# Autodesk Inventor assembly: 0.3rd Lawette - V3.0
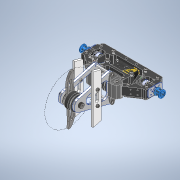
[picture p0: Inventor's stored thumbnail of the model, 180x180]
Saved by Autodesk Inventor 2022.1 (Build 261234020, 234B)
## iProperties
Created: 2022-05-21
Part Number: 0.3rd Lawette - V3.0
Document SubType Name: Assembly
Designer: Nathan Cai
Mass: 1280.13 g
Surface Area: 3794.37 cm^2
Volume: 778.123 cm^3
Density: 1.64515 g/cm^3
Author: Nathan Cai
## Documents named in this file (24)
- D:\Inventor\0.3rd Lawette - V3.0\0.3rd Lawette - V3.0.iam
- D:\Inventor\0.3rd Lawette - V3.0\RR Brushless\RR-Brushless-Planetary.iam
- D:\Inventor\0.3rd Lawette - V3.0\Tattu 4S 650mah\Tattu 650mah 4S.iam
- D:\Inventor\0.3rd Lawette - V3.0\BL20A.ipt
- D:\Inventor\0.3rd Lawette - V3.0\Talon 25A ESC.ipt
- D:\Inventor\0.3rd Lawette - V3.0\Receiver (FrSky RX6R).ipt
- D:\Inventor\0.3rd Lawette - V3.0\Fingertech Power Switch\Fingertech Mini Power Switch.iam
- D:\Inventor\0.3rd Lawette - V3.0\Weapon Assembly.iam
- D:\Inventor\0.3rd Lawette - V3.0\Hubs (Fingertech Twisthub).ipt
- D:\Inventor\0.3rd Lawette - V3.0\Chassis.ipt
- D:\Inventor\0.3rd Lawette - V3.0\Tires (Fingertech Foam Wheels).ipt
- D:\Inventor\0.3rd Lawette - V3.0\Standoff 1.5in.ipt
- D:\Inventor\0.3rd Lawette - V3.0\Cover (Inner).ipt
- D:\Inventor\0.3rd Lawette - V3.0\Cover (Inner Top).ipt
- C:\Users\NCai2\Documents\Inventor\Content Center Files\R2022\en-US\ANSI B18.6.3(27)\ANSI B18.6.3 - 6-32 UNC - 0.5(11).ipt
- D:\Inventor\0.3rd Lawette - V3.0\Cover (Outer).ipt
- C:\Users\NCai2\Documents\Inventor\Content Center Files\R2022\en-US\ANSI B18.6.3(27)\ANSI B18.6.3 - 6-32 UNC - 0.375(11).ipt
- C:\Users\NCai2\Documents\Inventor\Content Center Files\R2022\en-US\ANSI B18.6.3(27)\ANSI B18.6.3 - 6-32 UNC - 0.4375(11).ipt
- C:\Users\NCai2\Documents\Inventor\Content Center Files\R2022\en-US\SAE J773b\SAE J773b - No. 6. SAE Type L. Regular.ipt
- D:\Inventor\0.3rd Lawette - V3.0\Bracket.ipt
- C:\Users\NCai2\Documents\Inventor\Content Center Files\R2022\en-US\ANSI B18.6.3(27)\ANSI B18.6.3 - 6-32 UNC - 0.625(11).ipt
- C:\Users\NCai2\Documents\Inventor\Content Center Files\R2022\en-US\ANSI B18.6.3(27)\ANSI B18.6.3 - 6-32 UNC - 1(11).ipt
- D:\Inventor\0.3rd Lawette - V3.0\Motor Plates.ipt
- D:\Inventor\0.3rd Lawette - V3.0\Motor Plates - Rear Insert.ipt
## Components (67 placed, 23 different names)
1. RR-Brushless-Planetary:1 [sub-assembly] — Mate:1, Mate:4, Mate:7, Flush:4, Mate:27, Mate:147
2. RR-Brushless-Planetary:2 [sub-assembly] — Mate:1, Mate:5, Mate:6, Flush:5, Mate:149
3. Tattu 650mah 4S:1 [sub-assembly] — Mate:15, Flush:9
4. BL20A:1 — Mate:2, Flush:1, Flush:2, Mate:14, Flush:7, Mate:22
5. BL20A:2 — Mate:2, Flush:1, Flush:2, Mate:3, Flush:3, Flush:8
6. Talon 25A ESC:1 — Mate:13, Flush:6
7. Receiver (FrSky RX6R):1 — Mate:3, Flush:3, Flush:8
8. Fingertech Mini Power Switch:1 [sub-assembly] — Flush:12, Mate:25, Mate:26
9. Hubs (Fingertech Twisthub):1 — Mate:4, Mate:7, Mate:8, Mate:11
10. Hubs (Fingertech Twisthub):2 — Mate:5, Mate:6, Mate:9, Mate:10
11. Chassis:1 — Flush:4, Flush:5, Mate:13, Flush:6, Mate:14, Flush:7, Mate:15, Flush:9, Mate:16, Mate:17, Flush:10, Flush:12, Mate:22, Mate:23, Mate:24, Mate:25, Mate:26, Mate:27, Mate:28, Mate:31, Mate:91, Mate:92, Mate:113, Mate:114, Mate:115, Mate:116, Mate:117, Mate:118, Mate:119, Mate:120, Mate:121, Mate:146, Flush:20, Mate:148, Flush:21
12. Tires (Fingertech Foam Wheels):1 — Mate:9, Mate:10
13. Tires (Fingertech Foam Wheels):2 — Mate:8, Mate:11
14. Standoff 1.5in:1 — Mate:16, Flush:11, Mate:30, Mate:33, Mate:55, Mate:128
15. Standoff 1.5in:2 — Mate:17, Flush:10, Flush:11, Flush:15, Flush:16, Mate:52, Mate:126, Mate:132
16. Standoff 1.5in:5 — Mate:23, Flush:15, Mate:51
17. Standoff 1.5in:6 — Mate:24, Flush:16, Mate:29, Mate:32, Mate:54, Mate:130
18. Cover (Inner):1 — Mate:28, Mate:29, Mate:30, Mate:53
19. Cover (Inner Top):1 — Mate:31, Mate:32, Mate:33, Mate:34, Mate:35, Mate:36, Mate:37, Mate:38, Mate:39, Mate:40, Mate:41, Mate:42, Mate:43, Mate:44, Mate:45, Mate:46, Mate:47, Mate:48, Mate:49, Mate:50
20. Cover (Outer):1 — Mate:50, Mate:51, Mate:52, Mate:131, Mate:133, Mate:134, Mate:135, Mate:136, Mate:137
21. Cover (Outer):2 — Mate:53, Mate:54, Mate:55, Mate:122, Mate:123, Mate:124, Mate:125, Mate:127, Mate:129
22. Motor Plates:1 — Mate:113, Mate:114, Mate:115
23. Motor Plates:2 — Mate:116, Mate:117, Mate:118
24. Cross Recessed Truss Head Machine Screw - Type I - Inch No. 6 - 32 - 1/2:1 — Mate:34, Mate:35
25. Cross Recessed Truss Head Machine Screw - Type I - Inch No. 6 - 32 - 1/2:2 — Mate:36, Mate:37
26. Cross Recessed Truss Head Machine Screw - Type I - Inch No. 6 - 32 - 1/2:3 — Mate:38, Mate:39
27. Cross Recessed Truss Head Machine Screw - Type I - Inch No. 6 - 32 - 1/2:4 — Mate:40, Mate:41
28. Cross Recessed Truss Head Machine Screw - Type I - Inch No. 6 - 32 - 1/2:5 — Mate:42, Mate:43
29. Cross Recessed Truss Head Machine Screw - Type I - Inch No. 6 - 32 - 1/2:6 — Mate:44, Mate:45
30. Cross Recessed Truss Head Machine Screw - Type I - Inch No. 6 - 32 - 1/2:7 — Mate:46, Mate:47
31. Cross Recessed Truss Head Machine Screw - Type I - Inch No. 6 - 32 - 1/2:8 — Mate:48, Mate:49
32. Cross Recessed Truss Head Machine Screw - Type I - Inch No. 6 - 32 - 3/8:1 — Insert:17
33. Cross Recessed Truss Head Machine Screw - Type I - Inch No. 6 - 32 - 7/16:1 — Insert:13
34. Conical Spring Washer SAE J773b (Inch) No. 6. SAE Type L. Regular:17 — Mate:130, Mate:131, Insert:17
35. Conical Spring Washer SAE J773b (Inch) No. 6. SAE Type L. Regular:13 — Mate:122, Mate:123, Insert:13
36. Conical Spring Washer SAE J773b (Inch) No. 6. SAE Type L. Regular:14 — Mate:124, Mate:125, Insert:14
37. Conical Spring Washer SAE J773b (Inch) No. 6. SAE Type L. Regular:15 — Mate:126, Mate:127, Insert:15
38. Conical Spring Washer SAE J773b (Inch) No. 6. SAE Type L. Regular:16 — Mate:128, Mate:129, Insert:16
39. Cross Recessed Truss Head Machine Screw - Type I - Inch No. 6 - 32 - 7/16:2 — Insert:14
40. Cross Recessed Truss Head Machine Screw - Type I - Inch No. 6 - 32 - 7/16:3 — Insert:15
41. Cross Recessed Truss Head Machine Screw - Type I - Inch No. 6 - 32 - 7/16:4 — Insert:16
42. Conical Spring Washer SAE J773b (Inch) No. 6. SAE Type L. Regular:18 — Mate:132, Mate:133, Insert:18
43. Conical Spring Washer SAE J773b (Inch) No. 6. SAE Type L. Regular:19 — Mate:134, Mate:135, Insert:19
44. Conical Spring Washer SAE J773b (Inch) No. 6. SAE Type L. Regular:20 — Mate:136, Mate:137, Insert:20
45. Cross Recessed Truss Head Machine Screw - Type I - Inch No. 6 - 32 - 3/8:2 — Insert:18
46. Cross Recessed Truss Head Machine Screw - Type I - Inch No. 6 - 32 - 3/8:3 — Insert:19
47. Cross Recessed Truss Head Machine Screw - Type I - Inch No. 6 - 32 - 3/8:4 — Insert:20
48. Motor Plates - Rear Insert:1 — Mate:146, Mate:147, Flush:20
49. Motor Plates - Rear Insert:2 — Mate:148, Mate:149, Flush:21
50. Cross Recessed Truss Head Machine Screw - Type I - Inch No. 6 - 32 - 1:6 — Insert:24
51. Conical Spring Washer SAE J773b (Inch) No. 6. SAE Type L. Regular:24 — Mate:144, Mate:145, Insert:24
52. Cross Recessed Truss Head Machine Screw - Type I - Inch No. 6 - 32 - 1:3 — Insert:23
53. Conical Spring Washer SAE J773b (Inch) No. 6. SAE Type L. Regular:23 — Mate:142, Mate:143, Insert:23
54. Cross Recessed Truss Head Machine Screw - Type I - Inch No. 6 - 32 - 1:5 — Insert:22
55. Conical Spring Washer SAE J773b (Inch) No. 6. SAE Type L. Regular:22 — Mate:140, Mate:141, Insert:22
56. Cross Recessed Truss Head Machine Screw - Type I - Inch No. 6 - 32 - 1:1 — Insert:21
57. Conical Spring Washer SAE J773b (Inch) No. 6. SAE Type L. Regular:21 — Mate:138, Mate:139, Insert:21
58. Standoff 1.5in:7 — Mate:93, Mate:94, Mate:95, Mate:96
59. Standoff 1.5in:8 — Mate:90, Mate:97, Mate:98, Mate:99, Mate:100
60. Weapon Assembly:1 [sub-assembly] — Mate:101, Mate:102, Mate:103, Mate:104
61. Bracket:1 — Mate:101, Mate:103, Mate:104, Mate:138, Mate:139, Mate:140, Mate:141
62. Bracket:2 — Mate:90, Mate:91, Mate:92, Mate:102, Mate:142, Mate:143, Mate:144, Mate:145
63. Cross Recessed Truss Head Machine Screw - Type I - Inch No. 6 - 32 - 5/8:1 — Mate:93, Mate:94
64. Cross Recessed Truss Head Machine Screw - Type I - Inch No. 6 - 32 - 5/8:2 — Mate:95, Mate:96
65. Cross Recessed Truss Head Machine Screw - Type I - Inch No. 6 - 32 - 5/8:4 — Mate:99, Mate:100
66. Cross Recessed Truss Head Machine Screw - Type I - Inch No. 6 - 32 - 5/8:3 — Mate:97, Mate:98
67. Weapon Assembly:2 [sub-assembly] — Mate:119, Mate:120, Mate:121
## Relationships (136: Mate 105, Flush 19, Insert 12)
- Mate:1: RR-Brushless-Planetary:1 ↔ RR-Brushless-Planetary:2
- Mate:2: BL20A:1 ↔ BL20A:2
- Flush:1: BL20A:1 ↔ BL20A:2
- Flush:2: BL20A:1 ↔ BL20A:2
- Mate:3: BL20A:2 ↔ Receiver (FrSky RX6R):1
- Flush:3: BL20A:2 ↔ Receiver (FrSky RX6R):1
- Mate:4: RR-Brushless-Planetary:1 ↔ Hubs (Fingertech Twisthub):1
- Mate:5: RR-Brushless-Planetary:2 ↔ Hubs (Fingertech Twisthub):2
- Mate:6: RR-Brushless-Planetary:2 ↔ Hubs (Fingertech Twisthub):2
- Mate:7: RR-Brushless-Planetary:1 ↔ Hubs (Fingertech Twisthub):1
- Mate:8: Hubs (Fingertech Twisthub):1 ↔ Tires (Fingertech Foam Wheels):2
- Mate:9: Hubs (Fingertech Twisthub):2 ↔ Tires (Fingertech Foam Wheels):1
- Mate:10: Hubs (Fingertech Twisthub):2 ↔ Tires (Fingertech Foam Wheels):1
- Mate:11: Hubs (Fingertech Twisthub):1 ↔ Tires (Fingertech Foam Wheels):2
- Flush:4: RR-Brushless-Planetary:1 ↔ Chassis:1
- Flush:5: RR-Brushless-Planetary:2 ↔ Chassis:1
- Mate:13: Talon 25A ESC:1 ↔ Chassis:1
- Flush:6: Talon 25A ESC:1 ↔ Chassis:1
- Mate:14: BL20A:1 ↔ Chassis:1
- Flush:7: BL20A:1 ↔ Chassis:1
- Flush:8: BL20A:2 ↔ Receiver (FrSky RX6R):1
- Mate:15 (3.175 mm): Tattu 650mah 4S:1 ↔ Chassis:1
- Flush:9: Tattu 650mah 4S:1 ↔ Chassis:1
- Mate:16: Chassis:1 ↔ Standoff 1.5in:1
- Mate:17: Chassis:1 ↔ Standoff 1.5in:2
- Flush:10 (-6.35 mm): Chassis:1 ↔ Standoff 1.5in:2
- Flush:11: Standoff 1.5in:1 ↔ Standoff 1.5in:2
- Flush:12: Fingertech Mini Power Switch:1 ↔ Chassis:1
- [Mate]: Chassis:1 ↔ Standoff 1.5in:8
- [Mate]: Chassis:1 ↔ Standoff 1.5in:7
- Mate:22: BL20A:1 ↔ Chassis:1
- Mate:23: Chassis:1 ↔ Standoff 1.5in:5
- Mate:24: Chassis:1 ↔ Standoff 1.5in:6
- Flush:15: Standoff 1.5in:2 ↔ Standoff 1.5in:5
- Flush:16: Standoff 1.5in:2 ↔ Standoff 1.5in:6
- Mate:25: Fingertech Mini Power Switch:1 ↔ Chassis:1
- Mate:26: Fingertech Mini Power Switch:1 ↔ Chassis:1
- Mate:27: RR-Brushless-Planetary:1 ↔ Chassis:1
- Mate:28: Chassis:1 ↔ Cover (Inner):1
- Mate:29: Standoff 1.5in:6 ↔ Cover (Inner):1
- Mate:30: Standoff 1.5in:1 ↔ Cover (Inner):1
- Mate:31: Chassis:1 ↔ Cover (Inner Top):1
- Mate:32: Standoff 1.5in:6 ↔ Cover (Inner Top):1
- Mate:33: Standoff 1.5in:1 ↔ Cover (Inner Top):1
- Mate:34: Cover (Inner Top):1 ↔ Cross Recessed Truss Head Machine Screw - Type I - Inch No. 6 - 32 - 1/2:1
- Mate:35: Cover (Inner Top):1 ↔ Cross Recessed Truss Head Machine Screw - Type I - Inch No. 6 - 32 - 1/2:1
- Mate:36: Cover (Inner Top):1 ↔ Cross Recessed Truss Head Machine Screw - Type I - Inch No. 6 - 32 - 1/2:2
- Mate:37: Cover (Inner Top):1 ↔ Cross Recessed Truss Head Machine Screw - Type I - Inch No. 6 - 32 - 1/2:2
- Mate:38: Cover (Inner Top):1 ↔ Cross Recessed Truss Head Machine Screw - Type I - Inch No. 6 - 32 - 1/2:3
- Mate:39: Cover (Inner Top):1 ↔ Cross Recessed Truss Head Machine Screw - Type I - Inch No. 6 - 32 - 1/2:3
- Mate:40: Cover (Inner Top):1 ↔ Cross Recessed Truss Head Machine Screw - Type I - Inch No. 6 - 32 - 1/2:4
- Mate:41: Cover (Inner Top):1 ↔ Cross Recessed Truss Head Machine Screw - Type I - Inch No. 6 - 32 - 1/2:4
- Mate:42: Cover (Inner Top):1 ↔ Cross Recessed Truss Head Machine Screw - Type I - Inch No. 6 - 32 - 1/2:5
- Mate:43: Cover (Inner Top):1 ↔ Cross Recessed Truss Head Machine Screw - Type I - Inch No. 6 - 32 - 1/2:5
- Mate:44: Cover (Inner Top):1 ↔ Cross Recessed Truss Head Machine Screw - Type I - Inch No. 6 - 32 - 1/2:6
- Mate:45: Cover (Inner Top):1 ↔ Cross Recessed Truss Head Machine Screw - Type I - Inch No. 6 - 32 - 1/2:6
- Mate:46: Cover (Inner Top):1 ↔ Cross Recessed Truss Head Machine Screw - Type I - Inch No. 6 - 32 - 1/2:7
- Mate:47: Cover (Inner Top):1 ↔ Cross Recessed Truss Head Machine Screw - Type I - Inch No. 6 - 32 - 1/2:7
- Mate:48: Cover (Inner Top):1 ↔ Cross Recessed Truss Head Machine Screw - Type I - Inch No. 6 - 32 - 1/2:8
- Mate:49: Cover (Inner Top):1 ↔ Cross Recessed Truss Head Machine Screw - Type I - Inch No. 6 - 32 - 1/2:8
- Mate:50: Cover (Inner Top):1 ↔ Cover (Outer):1
- Mate:51: Standoff 1.5in:5 ↔ Cover (Outer):1
- Mate:52: Standoff 1.5in:2 ↔ Cover (Outer):1
- Mate:53: Cover (Inner):1 ↔ Cover (Outer):2
- Mate:54: Standoff 1.5in:6 ↔ Cover (Outer):2
- Mate:55: Standoff 1.5in:1 ↔ Cover (Outer):2
- [Mate]: Standoff 1.5in:7 ↔ Bracket:1
- [Flush]: Standoff 1.5in:7 ↔ Bracket:1
- [Flush] (-6.35 mm): Chassis:1 ↔ Standoff 1.5in:8
- [Flush]: Standoff 1.5in:7 ↔ Standoff 1.5in:8
- Mate:90: Standoff 1.5in:8 ↔ Bracket:2
- Mate:91: Chassis:1 ↔ Bracket:2
- Mate:92: Chassis:1 ↔ Bracket:2
- Mate:93: Standoff 1.5in:7 ↔ Cross Recessed Truss Head Machine Screw - Type I - Inch No. 6 - 32 - 5/8:1
- Mate:94: Standoff 1.5in:7 ↔ Cross Recessed Truss Head Machine Screw - Type I - Inch No. 6 - 32 - 5/8:1
- Mate:95: Standoff 1.5in:7 ↔ Cross Recessed Truss Head Machine Screw - Type I - Inch No. 6 - 32 - 5/8:2
- Mate:96: Standoff 1.5in:7 ↔ Cross Recessed Truss Head Machine Screw - Type I - Inch No. 6 - 32 - 5/8:2
- Mate:97: Standoff 1.5in:8 ↔ Cross Recessed Truss Head Machine Screw - Type I - Inch No. 6 - 32 - 5/8:3
- Mate:98: Standoff 1.5in:8 ↔ Cross Recessed Truss Head Machine Screw - Type I - Inch No. 6 - 32 - 5/8:3
- Mate:99: Standoff 1.5in:8 ↔ Cross Recessed Truss Head Machine Screw - Type I - Inch No. 6 - 32 - 5/8:4
- Mate:100: Standoff 1.5in:8 ↔ Cross Recessed Truss Head Machine Screw - Type I - Inch No. 6 - 32 - 5/8:4
- Mate:101: Weapon Assembly:1 ↔ Bracket:1
- Mate:102: Weapon Assembly:1 ↔ Bracket:2
- Mate:103: Weapon Assembly:1 ↔ Bracket:1
- Mate:104: Weapon Assembly:1 ↔ Bracket:1
- Mate:113: Chassis:1 ↔ Motor Plates:1
- Mate:114: Chassis:1 ↔ Motor Plates:1
- Mate:115: Chassis:1 ↔ Motor Plates:1
- Mate:116: Chassis:1 ↔ Motor Plates:2
- Mate:117: Chassis:1 ↔ Motor Plates:2
- Mate:118: Chassis:1 ↔ Motor Plates:2
- Mate:119: Chassis:1 ↔ Weapon Assembly:2
- Mate:120: Chassis:1 ↔ Weapon Assembly:2
- Mate:121 (6.35 mm): Chassis:1 ↔ Weapon Assembly:2
- Mate:122: Cover (Outer):2 ↔ Conical Spring Washer SAE J773b (Inch) No. 6. SAE Type L. Regular:13
- Mate:123: Cover (Outer):2 ↔ Conical Spring Washer SAE J773b (Inch) No. 6. SAE Type L. Regular:13
- Mate:124: Cover (Outer):2 ↔ Conical Spring Washer SAE J773b (Inch) No. 6. SAE Type L. Regular:14
- Mate:125: Cover (Outer):2 ↔ Conical Spring Washer SAE J773b (Inch) No. 6. SAE Type L. Regular:14
- Mate:126: Standoff 1.5in:2 ↔ Conical Spring Washer SAE J773b (Inch) No. 6. SAE Type L. Regular:15
- Mate:127: Cover (Outer):2 ↔ Conical Spring Washer SAE J773b (Inch) No. 6. SAE Type L. Regular:15
- Mate:128: Standoff 1.5in:1 ↔ Conical Spring Washer SAE J773b (Inch) No. 6. SAE Type L. Regular:16
- Mate:129: Cover (Outer):2 ↔ Conical Spring Washer SAE J773b (Inch) No. 6. SAE Type L. Regular:16
- Insert:13: Cross Recessed Truss Head Machine Screw - Type I - Inch No. 6 - 32 - 7/16:1 ↔ Conical Spring Washer SAE J773b (Inch) No. 6. SAE Type L. Regular:13
- Insert:14: Conical Spring Washer SAE J773b (Inch) No. 6. SAE Type L. Regular:14 ↔ Cross Recessed Truss Head Machine Screw - Type I - Inch No. 6 - 32 - 7/16:2
- Insert:15: Conical Spring Washer SAE J773b (Inch) No. 6. SAE Type L. Regular:15 ↔ Cross Recessed Truss Head Machine Screw - Type I - Inch No. 6 - 32 - 7/16:3
- Insert:16: Conical Spring Washer SAE J773b (Inch) No. 6. SAE Type L. Regular:16 ↔ Cross Recessed Truss Head Machine Screw - Type I - Inch No. 6 - 32 - 7/16:4
- Mate:130: Standoff 1.5in:6 ↔ Conical Spring Washer SAE J773b (Inch) No. 6. SAE Type L. Regular:17
- Mate:131: Cover (Outer):1 ↔ Conical Spring Washer SAE J773b (Inch) No. 6. SAE Type L. Regular:17
- Mate:132: Standoff 1.5in:2 ↔ Conical Spring Washer SAE J773b (Inch) No. 6. SAE Type L. Regular:18
- Mate:133: Cover (Outer):1 ↔ Conical Spring Washer SAE J773b (Inch) No. 6. SAE Type L. Regular:18
- Mate:134: Cover (Outer):1 ↔ Conical Spring Washer SAE J773b (Inch) No. 6. SAE Type L. Regular:19
- Mate:135: Cover (Outer):1 ↔ Conical Spring Washer SAE J773b (Inch) No. 6. SAE Type L. Regular:19
- Mate:136: Cover (Outer):1 ↔ Conical Spring Washer SAE J773b (Inch) No. 6. SAE Type L. Regular:20
- Mate:137: Cover (Outer):1 ↔ Conical Spring Washer SAE J773b (Inch) No. 6. SAE Type L. Regular:20
- Insert:17: Cross Recessed Truss Head Machine Screw - Type I - Inch No. 6 - 32 - 3/8:1 ↔ Conical Spring Washer SAE J773b (Inch) No. 6. SAE Type L. Regular:17
- Insert:18: Conical Spring Washer SAE J773b (Inch) No. 6. SAE Type L. Regular:18 ↔ Cross Recessed Truss Head Machine Screw - Type I - Inch No. 6 - 32 - 3/8:2
- Insert:19: Conical Spring Washer SAE J773b (Inch) No. 6. SAE Type L. Regular:19 ↔ Cross Recessed Truss Head Machine Screw - Type I - Inch No. 6 - 32 - 3/8:3
- Insert:20: Conical Spring Washer SAE J773b (Inch) No. 6. SAE Type L. Regular:20 ↔ Cross Recessed Truss Head Machine Screw - Type I - Inch No. 6 - 32 - 3/8:4
- Mate:138: Conical Spring Washer SAE J773b (Inch) No. 6. SAE Type L. Regular:21 ↔ Bracket:1
- Mate:139: Conical Spring Washer SAE J773b (Inch) No. 6. SAE Type L. Regular:21 ↔ Bracket:1
- Mate:140: Conical Spring Washer SAE J773b (Inch) No. 6. SAE Type L. Regular:22 ↔ Bracket:1
- Mate:141: Conical Spring Washer SAE J773b (Inch) No. 6. SAE Type L. Regular:22 ↔ Bracket:1
- Insert:21: Cross Recessed Truss Head Machine Screw - Type I - Inch No. 6 - 32 - 1:1 ↔ Conical Spring Washer SAE J773b (Inch) No. 6. SAE Type L. Regular:21
- Insert:22: Cross Recessed Truss Head Machine Screw - Type I - Inch No. 6 - 32 - 1:5 ↔ Conical Spring Washer SAE J773b (Inch) No. 6. SAE Type L. Regular:22
- Mate:142: Conical Spring Washer SAE J773b (Inch) No. 6. SAE Type L. Regular:23 ↔ Bracket:2
- Mate:143: Conical Spring Washer SAE J773b (Inch) No. 6. SAE Type L. Regular:23 ↔ Bracket:2
- Mate:144: Conical Spring Washer SAE J773b (Inch) No. 6. SAE Type L. Regular:24 ↔ Bracket:2
- Mate:145: Conical Spring Washer SAE J773b (Inch) No. 6. SAE Type L. Regular:24 ↔ Bracket:2
- Insert:23: Cross Recessed Truss Head Machine Screw - Type I - Inch No. 6 - 32 - 1:3 ↔ Conical Spring Washer SAE J773b (Inch) No. 6. SAE Type L. Regular:23
- Insert:24: Cross Recessed Truss Head Machine Screw - Type I - Inch No. 6 - 32 - 1:6 ↔ Conical Spring Washer SAE J773b (Inch) No. 6. SAE Type L. Regular:24
- Mate:146: Chassis:1 ↔ Motor Plates - Rear Insert:1
- Mate:147: RR-Brushless-Planetary:1 ↔ Motor Plates - Rear Insert:1
- Flush:20: Chassis:1 ↔ Motor Plates - Rear Insert:1
- Mate:148: Chassis:1 ↔ Motor Plates - Rear Insert:2
- Mate:149: RR-Brushless-Planetary:2 ↔ Motor Plates - Rear Insert:2
- Flush:21: Chassis:1 ↔ Motor Plates - Rear Insert:2
